# Autodesk Inventor assembly: Assembly
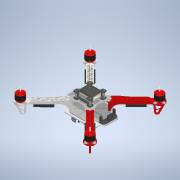
[picture p0: Inventor's stored thumbnail of the model, 180x180]
Saved by Autodesk Inventor 2020 (Build 240168000, 168)
## iProperties
Created: 2019-06-13
Part Number: Assembly
Document SubType Name: Assembly
Designer: amirt
Author: amirt
## Documents named in this file (14)
- C:\Users\amirt\Documents\Inventor\Drone\Assembly.iam
- C:\Users\amirt\Documents\Inventor\Drone\FrameParts\Frame.iam
- C:\Users\amirt\Documents\Inventor\Drone\Imported Components\Pixfalcon-Flight-Controller v1.ipt
- C:\Users\amirt\Documents\Inventor\Drone\Motor\Motor.iam
- C:\Users\amirt\Documents\Inventor\Drone\3DPrint\BatteryStopper.ipt
- C:\Users\amirt\Documents\Inventor\Drone\VibrationDampener.ipt
- C:\Users\amirt\Documents\Inventor\Drone\3DPrint\holder.ipt
- C:\Users\amirt\Documents\Inventor\Drone\3DPrint\cover.ipt
- C:\Users\amirt\Documents\Inventor\Drone\standoff.ipt
- C:\Users\amirt\Documents\Inventor\Drone\3DPrint\top.ipt
- C:\Users\amirt\Documents\Inventor\Drone\3DPrint\ESC.ipt
- C:\Users\amirt\Documents\Inventor\Drone\3DPrint\Battery.ipt
- C:\Users\amirt\Documents\Inventor\Drone\OdroidAssembly.iam
- C:\Users\amirt\Documents\Inventor\Drone\3DPrint\OdroidPlateSpacer.ipt
## Components (23 placed, 13 different names)
1. Frame:1 [sub-assembly] — Mate:2, Mate:3, Mate:4, Mate:5, Flush:1, Flush:3, Mate:6, Flush:4, Mate:7, Flush:6, Flush:7, Flush:8, Flush:9, Flush:16, Flush:18, Mate:17
2. Pixfalcon-Flight-Controller v1:1 — Mate:8, Flush:8, Flush:9, Mate:15, Mate:16
3. BatteryStopper:1 — Mate:5, Flush:1, Flush:17
4. VibrationDampener:1 — Flush:4, Mate:7, Flush:5
5. VibrationDampener:2 — Flush:3, Mate:6, Flush:5, Flush:6, Mate:8
6. holder:1 — Flush:7, Flush:12, Flush:13, Flush:14, Mate:9, Mate:10, Mate:11
7. cover:1 — Mate:15, Mate:16, Flush:19
8. standoff:1 — Flush:12, Flush:13, Flush:14
9. standoff:2 — Mate:11
10. standoff:3 — Mate:10, Flush:15
11. standoff:4 — Mate:9, Flush:19
12. top:1 — Flush:15
13. Battery:1 — Flush:17
14. OdroidAssembly:1 [sub-assembly] — Mate:18, Mate:19, Mate:20
15. OdroidPlateSpacer:1 — Flush:18, Mate:17, Mate:18, Mate:19, Mate:20
16. Motor:1 [sub-assembly] — Mate:3, Mate:4
17. Motor:2 [sub-assembly]
18. Motor:3 [sub-assembly]
19. Motor:4 [sub-assembly]
20. ESC:1 — Flush:16
21. ESC:2
22. ESC:3
23. ESC:4
## Component patterns: (4 elements, first: Motor:1), (4 elements, first: ESC:1)
## Relationships (32: Mate 16, Flush 16)
- Mate:2: Frame:1
- Mate:3: Frame:1 ↔ Motor:1
- Mate:4: Frame:1 ↔ Motor:1
- Mate:5: Frame:1 ↔ BatteryStopper:1
- Flush:1 (-1.5875 mm): Frame:1 ↔ BatteryStopper:1
- Flush:3: Frame:1 ↔ VibrationDampener:2
- Mate:6: Frame:1 ↔ VibrationDampener:2
- Flush:4: Frame:1 ↔ VibrationDampener:1
- Mate:7: Frame:1 ↔ VibrationDampener:1
- Flush:5: VibrationDampener:1 ↔ VibrationDampener:2
- Flush:6 (1.524 mm): Frame:1 ↔ VibrationDampener:2
- Flush:7: Frame:1 ↔ holder:1
- Mate:8: Pixfalcon-Flight-Controller v1:1 ↔ VibrationDampener:2
- Flush:8 (-5.0292 mm): Frame:1 ↔ Pixfalcon-Flight-Controller v1:1
- Flush:9 (-7.7724 mm): Frame:1 ↔ Pixfalcon-Flight-Controller v1:1
- Flush:12: holder:1 ↔ standoff:1
- Flush:13: holder:1 ↔ standoff:1
- Flush:14: holder:1 ↔ standoff:1
- Mate:9: holder:1 ↔ standoff:4
- Mate:10: holder:1 ↔ standoff:3
- Mate:11: holder:1 ↔ standoff:2
- Flush:15: standoff:3 ↔ top:1
- Flush:16: Frame:1 ↔ ESC:1
- Flush:17: BatteryStopper:1 ↔ Battery:1
- Mate:15: Pixfalcon-Flight-Controller v1:1 ↔ cover:1
- Mate:16: Pixfalcon-Flight-Controller v1:1 ↔ cover:1
- Flush:18: Frame:1 ↔ OdroidPlateSpacer:1
- Mate:17: Frame:1 ↔ OdroidPlateSpacer:1
- Mate:18: OdroidAssembly:1 ↔ OdroidPlateSpacer:1
- Mate:19 (-25.9969 mm): OdroidAssembly:1 ↔ OdroidPlateSpacer:1
- Mate:20 (-5.4737 mm): OdroidAssembly:1 ↔ OdroidPlateSpacer:1
- Flush:19: cover:1 ↔ standoff:4
